# Autodesk Inventor assembly: motherboard_asm
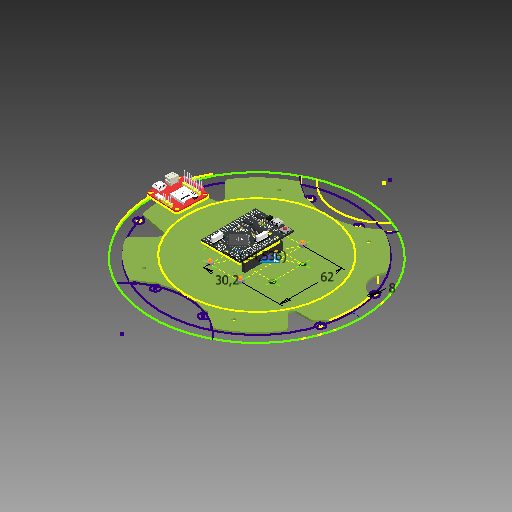
[picture p0: Inventor's stored thumbnail of the model, 512x512]
Saved by Autodesk Inventor 2020 (Build 240168000, 168)
## iProperties
Created: 2024-11-03
Part Number: motherboard_asm
Document SubType Name: Assembly
Designer: Ivan
Mass: 511.042 g
Surface Area: 867.217 cm^2
Volume: 101.76 cm^3
Density: 5.02202 g/cm^3
Author: Ivan
## Documents named in this file (13)
- C:\!projects\DASH-\3D\Dash-V1\motherboard\motherboard_asm.iam
- C:\!projects\DASH-\3D\Dash-V1\motherboard\motherboard.ipt
- C:\!projects\DASH-\3D\Dash-V1\boost.ipt
- C:\!projects\DASH-\3D\Dash-V1\step\m3_bolt\m3x8\Spacer Bolts_m3_bn_L5.ipt
- C:\!projects\DASH-\3D\Dash-V1\step\m3_bolt\Spacer Bolts_m3_bn_L5_ЗЕРКАЛО.ipt
- C:\!projects\DASH-\3D\Dash-V1\step\m3_bolt\Spacer Bolts_m3_bn_L5_ЗЕРКАЛО1.ipt
- C:\!projects\DASH-\3D\Dash-V1\step\m3_bolt\Spacer Bolts_m3_bn_L5_ЗЕРКАЛО_ЗЕРКАЛО.ipt
- C:\!projects\DASH-\3D\Dash-V1\step\mega\MEGA 2560 PRO (EMBED).iam
- C:\!projects\DASH-\3D\Dash-V1\step\SparkFun_9DoF_Razor_IMU\SparkFun 9DoF Razor IMU.ipt
- C:\!projects\DASH-\3D\Dash-V1\step\oled_0.96\Weewooday I2C OLED 0.96'' 128x64.iam
- C:\!projects\DASH-\3D\Dash-V1\step\HC\HC05_06.iam
- C:\!projects\DASH-\3D\Dash-V1\step\m3_bolt\m3x8\Гайка М3-6H ГОСТ 5927-70.ipt
- C:\!projects\DASH-\3D\Dash-V1\step\connectorJST\sol\jst2pins.iam
## Components (24 placed, 12 different names)
1. motherboard:1 — Совмещение:1, Совмещение:2, Угол:1, Вставка:1, Вставка:3, Вставка:4, Вставка:6, Вставка:7, Совмещение:4, Совмещение:5, Совмещение:6, Угол:3, Угол:4, Вставка:13, Вставка:14, Вставка:15, Вставка:16, Совмещение:7, Совмещение:8, Совмещение:9, Совмещение:10, Касательность:1, Касательность:2, Совмещение:13, Совмещение:14
2. MEGA 2560 PRO (EMBED):1 [sub-assembly] — Угол:2, Совмещение:5, Заподлицо:1, Угол:3
3. SparkFun 9DoF Razor IMU:1 — Заподлицо:1
4. Weewooday I2C OLED 0.96'' 128x64:1 [sub-assembly] — Совмещение:6, Угол:4
5. HC05_06:1 [sub-assembly] — Совмещение:4, Угол:2
6. jst2pins:1 [sub-assembly] — Совмещение:10, Угол:7, Касательность:1, Симметрия:1, Совмещение:11, Совмещение:12
7. jst2pins:2 [sub-assembly] — Совмещение:7, Симметрия:2
8. jst2pins:3 [sub-assembly] — Совмещение:9, Угол:5, Касательность:2, Симметрия:1, Симметрия:2
9. jst2pins:4 [sub-assembly] — Совмещение:8, Совмещение:11, Совмещение:12
10. jst2pins:5 [sub-assembly] — Совмещение:14, Угол:8, Симметрия:3, Заподлицо:2, Заподлицо:3
11. jst2pins:6 [sub-assembly] — Совмещение:13, Симметрия:3, Заподлицо:2
12. Spacer Bolts_m3_bn_L5:4 — Вставка:4
13. Spacer Bolts_m3_bn_L5:3 — Вставка:6, Вставка:12
14. Spacer Bolts_m3_bn_L5:2 — Вставка:1
15. Spacer Bolts_m3_bn_L5:1 — Вставка:3, Вставка:11
16. boost:1 — Вставка:11, Вставка:12, Заподлицо:3
17. Spacer Bolts_m3_bn_L5:7 — Вставка:7
18. Spacer Bolts_m3_bn_L5_ЗЕРКАЛО:3
19. Spacer Bolts_m3_bn_L5_ЗЕРКАЛО1:3
20. Spacer Bolts_m3_bn_L5_ЗЕРКАЛО_ЗЕРКАЛО:3
21. Гайка М3-6H ГОСТ 5927-70:1 — Вставка:14
22. Гайка М3-6H ГОСТ 5927-70:2 — Вставка:16
23. Гайка М3-6H ГОСТ 5927-70:3 — Вставка:13
24. Гайка М3-6H ГОСТ 5927-70:4 — Вставка:15
## Relationships (39: Mate 13, Insert 11, Angle 7, Flush 3, Symmetry 3, Tangent 2)
- Совмещение:1 [Mate]: motherboard:1
- Совмещение:2 [Mate]: motherboard:1
- Угол:1 [Angle] (-45 deg): motherboard:1
- Вставка:1 [Insert]: motherboard:1 ↔ Spacer Bolts_m3_bn_L5:2
- Вставка:3 [Insert]: motherboard:1 ↔ Spacer Bolts_m3_bn_L5:1
- Вставка:4 [Insert]: motherboard:1 ↔ Spacer Bolts_m3_bn_L5:4
- Вставка:6 [Insert]: motherboard:1 ↔ Spacer Bolts_m3_bn_L5:3
- Вставка:7 [Insert] (5 mm): motherboard:1 ↔ Spacer Bolts_m3_bn_L5:7
- Совмещение:4 [Mate]: motherboard:1 ↔ HC05_06:1
- Угол:2 [Angle] (180 deg): MEGA 2560 PRO (EMBED):1 ↔ HC05_06:1
- Вставка:11 [Insert]: Spacer Bolts_m3_bn_L5:1 ↔ boost:1
- Вставка:12 [Insert]: Spacer Bolts_m3_bn_L5:3 ↔ boost:1
- Совмещение:5 [Mate]: motherboard:1 ↔ MEGA 2560 PRO (EMBED):1
- Совмещение:6 [Mate] (0.1 mm): motherboard:1 ↔ Weewooday I2C OLED 0.96'' 128x64:1
- Заподлицо:1 [Flush]: MEGA 2560 PRO (EMBED):1 ↔ SparkFun 9DoF Razor IMU:1
- Угол:3 [Angle] (90 deg): motherboard:1 ↔ MEGA 2560 PRO (EMBED):1
- Угол:4 [Angle] (135 deg): motherboard:1 ↔ Weewooday I2C OLED 0.96'' 128x64:1
- Вставка:13 [Insert]: motherboard:1 ↔ Гайка М3-6H ГОСТ 5927-70:3
- Вставка:14 [Insert]: motherboard:1 ↔ Гайка М3-6H ГОСТ 5927-70:1
- Вставка:15 [Insert]: motherboard:1 ↔ Гайка М3-6H ГОСТ 5927-70:4
- Вставка:16 [Insert]: motherboard:1 ↔ Гайка М3-6H ГОСТ 5927-70:2
- Совмещение:7 [Mate]: motherboard:1 ↔ jst2pins:2
- Совмещение:8 [Mate]: motherboard:1 ↔ jst2pins:4
- Совмещение:9 [Mate]: motherboard:1 ↔ jst2pins:3
- Совмещение:10 [Mate]: motherboard:1 ↔ jst2pins:1
- Угол:5 [Angle] (45 deg): jst2pins:3
- Угол:7 [Angle] (45 deg): jst2pins:1
- Касательность:1 [Tangent] (5 mm): motherboard:1 ↔ jst2pins:1
- Касательность:2 [Tangent] (5 mm): motherboard:1 ↔ jst2pins:3
- Симметрия:1 [Symmetry]: jst2pins:1 ↔ jst2pins:3
- Симметрия:2 [Symmetry]: jst2pins:2 ↔ jst2pins:3
- Совмещение:11 [Mate] (4 mm): jst2pins:1 ↔ jst2pins:4
- Совмещение:12 [Mate] (2 mm): jst2pins:1 ↔ jst2pins:4
- Совмещение:13 [Mate]: motherboard:1 ↔ jst2pins:6
- Совмещение:14 [Mate]: motherboard:1 ↔ jst2pins:5
- Угол:8 [Angle] (0 deg): jst2pins:5
- Симметрия:3 [Symmetry]: jst2pins:5 ↔ jst2pins:6
- Заподлицо:2 [Flush]: jst2pins:5 ↔ jst2pins:6
- Заподлицо:3 [Flush] (31.25 mm): jst2pins:5 ↔ boost:1
